# Autodesk Inventor assembly: power button
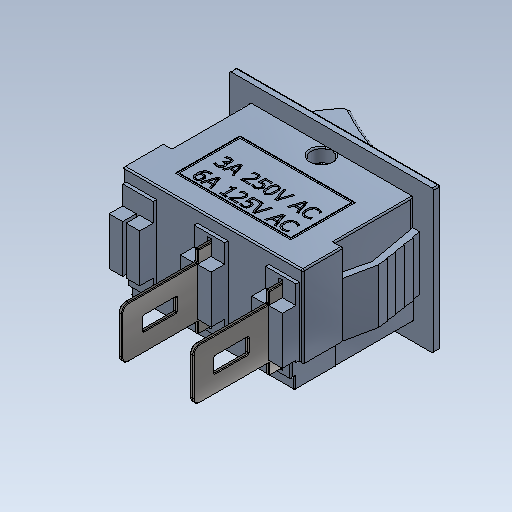
[picture p0: Inventor's stored thumbnail of the model, 512x512]
Saved by Autodesk Inventor 2025 (Build 290162000, 162)
## iProperties
Created: 2017-03-16
Part Number: power button
Document SubType Name: Assembly
Designer: Win10
Author: Win10
## Documents named in this file (7)
- C:\Users\HP\Downloads\Compressed\power-switch-power-button-1.snapshot.2\power button.iam
- C:\Users\HP\Downloads\Compressed\power-switch-power-button-1.snapshot.2\power buton ust.ipt
- C:\Users\HP\Downloads\Compressed\power-switch-power-button-1.snapshot.2\ic.ipt
- C:\Users\HP\Downloads\Compressed\power-switch-power-button-1.snapshot.2\metal göbek.ipt
- C:\Users\HP\Downloads\Compressed\power-switch-power-button-1.snapshot.2\metal uc.ipt
- C:\Users\HP\Downloads\Compressed\power-switch-power-button-1.snapshot.2\metal uc2.ipt
- C:\Users\HP\Downloads\Compressed\power-switch-power-button-1.snapshot.2\plastik kafa.ipt
## Components (6 placed, 6 different names)
1. power buton ust:1 — Mate:1, Mate:2, Mate:3, Mate:4, Flush:1, Mate:5
2. ic:1 — Mate:1, Mate:2, Mate:7, Mate:8
3. metal göbek:1 — Mate:6, Mate:9, Mate:10
4. metal uc:1 — Mate:3, Mate:4, Flush:1, Flush:2, Flush:3, Mate:6, Mate:9, Mate:10
5. metal uc2:1 — Mate:5, Flush:2, Flush:3
6. plastik kafa:1 — Mate:7, Mate:8
## Relationships (13: Mate 10, Flush 3)
- Mate:1: power buton ust:1 ↔ ic:1
- Mate:2 (0.25 mm): power buton ust:1 ↔ ic:1
- Mate:3: power buton ust:1 ↔ metal uc:1
- Mate:4 (0.25 mm): power buton ust:1 ↔ metal uc:1
- Flush:1 (-0.5 mm): power buton ust:1 ↔ metal uc:1
- Mate:5: power buton ust:1 ↔ metal uc2:1
- Flush:2: metal uc:1 ↔ metal uc2:1
- Flush:3: metal uc:1 ↔ metal uc2:1
- Mate:6: metal göbek:1 ↔ metal uc:1
- Mate:7: ic:1 ↔ plastik kafa:1
- Mate:8: ic:1 ↔ plastik kafa:1
- Mate:9 (0.4 mm): metal göbek:1 ↔ metal uc:1
- Mate:10 (0.4 mm): metal göbek:1 ↔ metal uc:1
